# Autodesk Inventor assembly: Intake
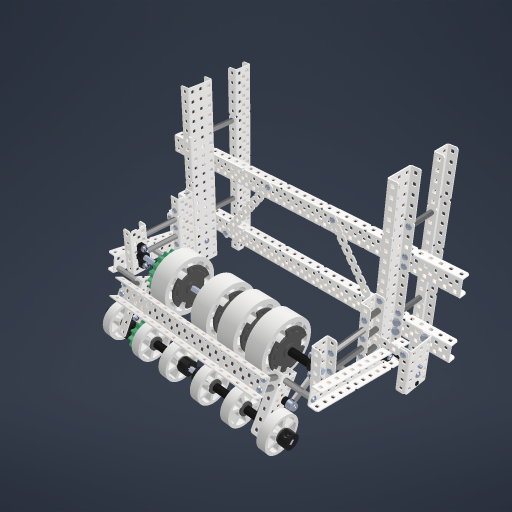
[picture p0: Inventor's stored thumbnail of the model, 512x512]
Saved by Autodesk Inventor 2023 (Build 270158000, 158)
## iProperties
Created: 2022-09-02
Part Number: Intake
Document SubType Name: Assembly
Designer: alex
Author: alex
## Documents named in this file (43)
- C:\Users\alex\Documents\GitHub\4067X_spin_up_cad\Mechanism\Intake.iam
- C:\Users\alex\Documents\GitHub\4067X_spin_up_cad\Library\Structure\Standoff\Standoff 1.00.ipt
- C:\Users\alex\Documents\GitHub\4067X_spin_up_cad\Library\Structure\Standoff.ipt
- C:\Users\alex\Documents\GitHub\4067X_spin_up_cad\Library\Structure\Hardware\Screw Steel - Star\SScrew Star Smooth .290.ipt
- C:\Users\alex\Documents\GitHub\4067X_spin_up_cad\Library\Structure\Hardware\Screw Steel - Star.ipt
- C:\Users\alex\Documents\GitHub\4067X_spin_up_cad\Library\Structure\Standoff\Standoff .50.ipt
- C:\Users\alex\Documents\GitHub\4067X_spin_up_cad\Library\Motion\Spacers\Spacer Nylon .375 OD.ipt
- C:\Users\alex\Documents\GitHub\4067X_spin_up_cad\Library\Structure\Hardware\Nut Keps.ipt
- C:\Users\alex\Documents\GitHub\4067X_spin_up_cad\Library\Structure\Hardware\Screw Steel - Star\SScrew Star Smooth .375.ipt
- C:\Users\alex\Documents\GitHub\4067X_spin_up_cad\Library\Structure\C-Channels\Aluminum 1x3x1\Alu C 1x3x1x20.ipt
- C:\Users\alex\Documents\GitHub\4067X_spin_up_cad\Library\Structure\C-Channels\Aluminum 1x3x1\Alu C 1x3x1x5.ipt
- C:\Users\alex\Documents\GitHub\4067X_spin_up_cad\Library\Structure\C-Channels\Aluminum 1x2x1\Alu C 1x2x1x35.ipt
- C:\Users\alex\Documents\GitHub\4067X_spin_up_cad\Library\Structure\Plates\Aluminum\VEX Plates\Alu Plate VEX 1x11.ipt
- C:\Users\alex\Documents\GitHub\4067X_spin_up_cad\Library\Structure\Standoff\Standoff 2.00.ipt
- C:\Users\alex\Documents\GitHub\4067X_spin_up_cad\Library\Structure\C-Channels\Aluminum 1x2x1\Alu C 1x2x1x5.ipt
- C:\Users\alex\Documents\GitHub\4067X_spin_up_cad\Library\Structure\C-Channels\Aluminum 1x2x1\Alu C 1x2x1x7.ipt
- C:\Users\alex\Documents\GitHub\4067X_spin_up_cad\Library\Structure\Standoff\Standoff .75.ipt
- C:\Users\alex\Documents\GitHub\4067X_spin_up_cad\Library\Motion\Spacers\Spacer Nylon .375 OD\NSpacer .375 OD x .125.ipt
- C:\Users\alex\Documents\GitHub\4067X_spin_up_cad\Library\Motion\Shaft HS\HS Bearing Flat.ipt
- C:\Users\alex\Documents\GitHub\4067X_spin_up_cad\Library\Structure\Hardware\Nut Thin Nylock.ipt
- C:\Users\alex\Documents\GitHub\4067X_spin_up_cad\Library\Structure\Hardware\Screw Steel - Star\SScrew Star Smooth .500.ipt
- C:\Users\alex\Documents\GitHub\4067X_spin_up_cad\Library\Motion\Shaft HS\Shaft HS\Shaft HS 12.0 in.ipt
- C:\Users\alex\Documents\GitHub\4067X_spin_up_cad\Library\Motion\Shaft HS\Shaft HS.ipt
- C:\Users\alex\Documents\GitHub\4067X_spin_up_cad\Library\Motion\Shaft HS\HS Spacer.ipt
- C:\Users\alex\Documents\GitHub\4067X_spin_up_cad\3FlexWheel.iam
- C:\Users\alex\Documents\GitHub\4067X_spin_up_cad\Library\Motion\Shaft HS\HS Spacer\HSpacer .2500.ipt
- C:\Users\alex\Documents\GitHub\4067X_spin_up_cad\Library\Motion\Sprockets\HS 18T Sprocket, No Insert.ipt
- C:\Users\alex\Documents\GitHub\4067X_spin_up_cad\Library\Structure\Hardware\Screw Steel - Star\SScrew Star Smooth 2.250.ipt
- C:\Users\alex\Documents\GitHub\4067X_spin_up_cad\Mechanism\FloatingIntake.iam
- C:\Users\alex\Documents\GitHub\4067X_spin_up_cad\Library\Motion\Spacers\Spacer Nylon .375 OD\NSpacer .375 OD x .375.ipt
- C:\Users\alex\Documents\GitHub\4067X_spin_up_cad\Library\Motion\Spacers\Washer Steel\SWasher .375 OD x .015625.ipt
- C:\Users\alex\Documents\GitHub\4067X_spin_up_cad\Library\Motion\Spacers\Washer Steel.ipt
- C:\Users\alex\Documents\GitHub\4067X_spin_up_cad\Library\Motion\1-Post Bearing Flat Hex Retainer.ipt
- C:\Users\alex\Documents\GitHub\4067X_spin_up_cad\Library\Structure\Hardware\Nut Nylock.ipt
- C:\Users\alex\Documents\GitHub\4067X_spin_up_cad\Library\Motion\Spacers\Spacer Nylon .375 OD\NSpacer .375 OD x .500.ipt
- C:\Users\alex\Documents\GitHub\4067X_spin_up_cad\Library\Motion\Spacers\Washer Teflon\TWasher .375 OD x .06250.ipt
- C:\Users\alex\Documents\GitHub\4067X_spin_up_cad\Library\Motion\Spacers\Washer Teflon.ipt
- C:\Users\alex\Documents\GitHub\4067X_spin_up_cad\Library\Structure\Plates\Aluminum\VEX Plates\Alu Plate VEX 1x4.ipt
- C:\Users\alex\Documents\GitHub\4067X_spin_up_cad\Library\Motion\Shaft HS\HS Shaft Collar.ipt
- C:\Users\alex\Documents\GitHub\4067X_spin_up_cad\Library\Motion\Shaft HS\HS Spacer\HSpacer .5000.ipt
- C:\Users\alex\Documents\GitHub\4067X_spin_up_cad\Library\Motion\Shaft HS\HS Spacer\HSpacer .1250.ipt
- C:\Users\alex\Documents\GitHub\4067X_spin_up_cad\Library\Structure\C-Channels\Aluminum 1x2x1\Alu C 1x2x1x21.ipt
- C:\Users\alex\Documents\GitHub\4067X_spin_up_cad\Library\Structure\Hardware\Screw Steel - Star\SScrew Star Smooth .750.ipt
## Components (157 placed, 35 different names)
1. Alu C 1x3x1x5:1 — Insert:107, Insert:108, Insert:230, Insert:244, Insert:245, Insert:437, Mate:68, Insert:438, Insert:444
2. Alu C 1x2x1x35:1 — Insert:107, Insert:108, Insert:150, Insert:151, Insert:218, Insert:219, Insert:236, Insert:237, Insert:400, Insert:401, Insert:419, Insert:420, Insert:448, Insert:449, Insert:458, Insert:459, Insert:465, Insert:469, Insert:475, Insert:478
3. Standoff 1.00:16 — Insert:110, Insert:404
4. Standoff .50:17 — Insert:110, Insert:496
5. Standoff 1.00:18 — Insert:405
6. Standoff .50:19 — Insert:497
7. Standoff 1.00:20 — Insert:454
8. Standoff .50:21 — Insert:500
9. Standoff 1.00:22 — Insert:455
10. Standoff .50:23 — Insert:501
11. Alu C 1x3x1x5:2 — Insert:150, Insert:151, Insert:217, Insert:220, Insert:221, Insert:428, Mate:67, Insert:429, Insert:439
12. Nut Keps:12 — Insert:217
13. SScrew Star Smooth .290:52 — Insert:218
14. SScrew Star Smooth .290:53 — Insert:219
15. Nut Keps:13 — Insert:220
16. Nut Keps:14 — Insert:221
17. Nut Keps:17 — Insert:230
18. SScrew Star Smooth .290:62 — Insert:236
19. SScrew Star Smooth .290:63 — Insert:237
20. Nut Keps:21 — Insert:244
21. Nut Keps:22 — Insert:245
22. Alu C 1x2x1x35:2 — Insert:417, Insert:418, Insert:466, Insert:467, Insert:470, Insert:476, Insert:477, Insert:481, Insert:482
23. SScrew Star Smooth .290:86 — Insert:456
24. SScrew Star Smooth .290:90 — Insert:407
25. SScrew Star Smooth .290:91 — Insert:406
26. Alu C 1x2x1x5:2 — Insert:334, Insert:335, Insert:338, Insert:339, Insert:488, Mate:72, Insert:489, Insert:490
27. Standoff 2.00:27 — Insert:334, Insert:382
28. Standoff 2.00:28 — Insert:335, Insert:381
29. SScrew Star Smooth .290:102 — Insert:338
30. SScrew Star Smooth .290:103 — Insert:339
31. Alu C 1x2x1x7:1 — Insert:345, Insert:346, Insert:347, Insert:348, Insert:349, Insert:358, Insert:359, Insert:360, Insert:361, Insert:362, Insert:381, Insert:382, Insert:422, Insert:423, Mate:69
32. SScrew Star Smooth .290:106 — Insert:345
33. SScrew Star Smooth .290:107 — Insert:346
34. Standoff .75:29 — Insert:347, Insert:355
35. Standoff .75:30 — Insert:348, Insert:356
36. Standoff .75:31 — Insert:349, Insert:357
37. NSpacer .375 OD x .125:13 — Insert:355
38. NSpacer .375 OD x .125:14 — Insert:356
39. NSpacer .375 OD x .125:15 — Insert:357
40. SScrew Star Smooth .375:111 — Insert:358
41. SScrew Star Smooth .375:112 — Insert:359
42. SScrew Star Smooth .375:113 — Insert:360
43. SScrew Star Smooth .290:114 — Insert:361
44. SScrew Star Smooth .290:115 — Insert:362
45. Alu C 1x2x1x5:3 — Insert:485, Mate:71, Insert:486, Insert:487, Flush:1
46. Standoff 2.00:32 — Insert:384
47. Standoff 2.00:33 — Insert:383
48. SScrew Star Smooth .290:116
49. SScrew Star Smooth .290:117
50. Alu C 1x2x1x7:2 — Insert:383, Insert:384, Insert:402, Insert:403, Mate:70
51. SScrew Star Smooth .290:118
52. SScrew Star Smooth .290:119
53. Standoff .75:34
54. Standoff .75:35
55. Standoff .75:36
56. NSpacer .375 OD x .125:16
57. NSpacer .375 OD x .125:17
58. NSpacer .375 OD x .125:18
59. SScrew Star Smooth .375:120
60. SScrew Star Smooth .375:121
61. SScrew Star Smooth .375:122
62. SScrew Star Smooth .290:123
63. SScrew Star Smooth .290:124
64. Shaft HS 12.0 in:1 — Mate:43, Angle:1, Angle:2, Mate:47, Mate:50, Mate:51, Mate:53, Angle:3, Mate:57, Angle:4, Mate:58, Angle:5, Mate:73, Flush:1, Mate:74
65. 3FlexWheel:1 [sub-assembly] — Mate:43, Angle:1, Mate:48, Mate:76
66. 3FlexWheel:2 [sub-assembly] — Angle:2, Mate:49, Mate:50, Mate:52
67. HSpacer .2500:2 — Mate:47, Mate:48, Mate:49
68. HSpacer .2500:3 — Mate:51, Mate:52, Mate:54
69. 3FlexWheel:3 [sub-assembly] — Mate:53, Angle:3, Mate:54
70. 3FlexWheel:4 [sub-assembly] — Mate:58, Angle:5, Mate:59
71. HS 18T Sprocket, No Insert:1 — Mate:57, Angle:4, Mate:59, Flush:2, Mate:75
72. Alu C 1x3x1x20:3 — Insert:400, Insert:401, Insert:402, Insert:403, Insert:404, Insert:405, Insert:406, Insert:407, Insert:408, Insert:409, Insert:410, Insert:411, Insert:412, Insert:413, Insert:414, Insert:416, Insert:460, Insert:461, Insert:467, Insert:468
73. Nut Keps:41 — Insert:408
74. Nut Keps:42 — Insert:409
75. SScrew Star Smooth .290:129 — Insert:410
76. SScrew Star Smooth .290:130 — Insert:411
77. SScrew Star Smooth .290:131 — Insert:412
78. SScrew Star Smooth 2.250:132 — Insert:413
79. Nut Keps:43 — Insert:414, Insert:433
80. SScrew Star Smooth .290:134 — Insert:416
81. Nut Keps:44 — Insert:417
82. Nut Keps:45 — Insert:418
83. Alu C 1x3x1x20:4 — Insert:419, Insert:420, Insert:421, Insert:422, Insert:423, Insert:424, Mate:66, Insert:446, Insert:450, Insert:451, Insert:452, Insert:453, Insert:454, Insert:455, Insert:456, Insert:457, Insert:462, Insert:463, Insert:464, Insert:479, Insert:480
84. SScrew Star Smooth 2.250:135 — Insert:421, Mate:65
85. Nut Keps:46 — Insert:424, Insert:425
86. FloatingIntake:1 [sub-assembly] — Mate:65, Mate:66, Insert:430, Insert:435, Flush:2
87. NSpacer .375 OD x .375:19 — Insert:425, Insert:426
88. SWasher .375 OD x .015625:1 — Insert:426
89. 1-Post Bearing Flat Hex Retainer:1 — Insert:428, Mate:67
90. Nut Nylock:1
91. SScrew Star Smooth .375:136 — Insert:429
92. NSpacer .375 OD x .500:20 — Insert:430, Insert:431
93. NSpacer .375 OD x .375:21 — Insert:431
94. NSpacer .375 OD x .375:22 — Insert:433
95. SWasher .375 OD x .015625:2
96. NSpacer .375 OD x .500:23 — Insert:435
97. NSpacer .375 OD x .375:24
98. 1-Post Bearing Flat Hex Retainer:2 — Insert:437, Mate:68
99. Nut Nylock:2
100. SScrew Star Smooth .375:137 — Insert:438
101. TWasher .375 OD x .06250:1 — Insert:439, Insert:440
102. Alu Plate VEX 1x4:1 — Insert:440, Mate:69, Insert:441, Insert:447
103. SScrew Star Smooth .375:138 — Insert:441
104. TWasher .375 OD x .06250:2 — Insert:444
105. Alu Plate VEX 1x4:2 — Mate:70
106. SScrew Star Smooth .375:139
107. Nut Keps:47 — Insert:446
108. SScrew Star Smooth .375:140 — Insert:447
109. SScrew Star Smooth .290:141 — Insert:448
110. SScrew Star Smooth .290:142 — Insert:449
111. Nut Keps:48 — Insert:450
112. Nut Keps:49 — Insert:451
113. Nut Keps:50 — Insert:452
114. Nut Keps:51 — Insert:453
115. SScrew Star Smooth .290:143 — Insert:457
116. SScrew Star Smooth .290:144 — Insert:458
117. SScrew Star Smooth .290:145 — Insert:459
118. Nut Keps:52 — Insert:460
119. Nut Keps:53 — Insert:461
120. SScrew Star Smooth .290:146 — Insert:462
121. SScrew Star Smooth .290:147 — Insert:463
122. SScrew Star Smooth .290:148 — Insert:464
123. Alu Plate VEX 1x11:3 — Insert:465, Insert:466, Insert:471, Insert:472
124. SScrew Star Smooth .290:149 — Insert:468
125. Alu Plate VEX 1x11:4 — Insert:469, Insert:470, Insert:473, Insert:474
126. SScrew Star Smooth .290:150 — Insert:471
127. SScrew Star Smooth .290:151 — Insert:472
128. SScrew Star Smooth .290:152 — Insert:473
129. SScrew Star Smooth .290:153 — Insert:474
130. Nut Keps:54 — Insert:475
131. Nut Keps:55 — Insert:476
132. Nut Keps:56 — Insert:477
133. Nut Keps:57 — Insert:478
134. SScrew Star Smooth .290:154 — Insert:479
135. SScrew Star Smooth .290:155 — Insert:480
136. Nut Keps:58 — Insert:481
137. Nut Keps:59 — Insert:482
138. HS Bearing Flat:3 — Insert:485, Mate:71, Insert:493
139. Nut Thin Nylock:5
140. Nut Thin Nylock:6
141. SScrew Star Smooth .500:156 — Insert:486
142. SScrew Star Smooth .500:157 — Insert:487
143. HS Bearing Flat:4 — Insert:488, Mate:72, Mate:73, Insert:491, Insert:492
144. SScrew Star Smooth .500:158 — Insert:489
145. SScrew Star Smooth .500:159 — Insert:490
146. Nut Thin Nylock:7 — Insert:491
147. Nut Thin Nylock:8 — Insert:492
148. HS Shaft Collar:1 — Mate:74, Mate:75
149. HSpacer .5000:4 — Insert:493, Insert:494
150. HSpacer .5000:5 — Insert:494, Insert:495
151. HSpacer .1250:6 — Insert:495, Mate:76
152. Alu C 1x2x1x21:1 — Insert:496, Insert:497, Insert:498, Insert:499
153. SScrew Star Smooth .750:160 — Insert:498
154. SScrew Star Smooth .750:161 — Insert:499
155. Alu C 1x2x1x21:2 — Insert:500, Insert:501, Insert:502, Insert:503
156. SScrew Star Smooth .750:162 — Insert:502
157. SScrew Star Smooth .750:163 — Insert:503
## Relationships (189: Insert 158, Mate 24, Angle 5, Flush 2)
- Insert:107: Alu C 1x3x1x5:1 ↔ Alu C 1x2x1x35:1
- Insert:108: Alu C 1x3x1x5:1 ↔ Alu C 1x2x1x35:1
- Insert:110: Standoff 1.00:16 ↔ Standoff .50:17
- [Insert]: Standoff 1.00:18 ↔ Standoff .50:19
- [Insert]: Standoff 1.00:20 ↔ Standoff .50:21
- [Insert]: Standoff 1.00:22 ↔ Standoff .50:23
- Insert:150: Alu C 1x2x1x35:1 ↔ Alu C 1x3x1x5:2
- Insert:151: Alu C 1x2x1x35:1 ↔ Alu C 1x3x1x5:2
- Insert:217: Alu C 1x3x1x5:2 ↔ Nut Keps:12
- Insert:218: Alu C 1x2x1x35:1 ↔ SScrew Star Smooth .290:52
- Insert:219: Alu C 1x2x1x35:1 ↔ SScrew Star Smooth .290:53
- Insert:220: Alu C 1x3x1x5:2 ↔ Nut Keps:13
- Insert:221: Alu C 1x3x1x5:2 ↔ Nut Keps:14
- Insert:230: Alu C 1x3x1x5:1 ↔ Nut Keps:17
- Insert:236: Alu C 1x2x1x35:1 ↔ SScrew Star Smooth .290:62
- Insert:237: Alu C 1x2x1x35:1 ↔ SScrew Star Smooth .290:63
- Insert:244: Alu C 1x3x1x5:1 ↔ Nut Keps:21
- Insert:245: Alu C 1x3x1x5:1 ↔ Nut Keps:22
- Insert:334: Alu C 1x2x1x5:2 ↔ Standoff 2.00:27
- Insert:335: Alu C 1x2x1x5:2 ↔ Standoff 2.00:28
- Insert:338: Alu C 1x2x1x5:2 ↔ SScrew Star Smooth .290:102
- Insert:339: Alu C 1x2x1x5:2 ↔ SScrew Star Smooth .290:103
- Insert:345: Alu C 1x2x1x7:1 ↔ SScrew Star Smooth .290:106
- Insert:346: Alu C 1x2x1x7:1 ↔ SScrew Star Smooth .290:107
- Insert:347: Alu C 1x2x1x7:1 ↔ Standoff .75:29
- Insert:348: Alu C 1x2x1x7:1 ↔ Standoff .75:30
- Insert:349: Alu C 1x2x1x7:1 ↔ Standoff .75:31
- Insert:355: Standoff .75:29 ↔ NSpacer .375 OD x .125:13
- Insert:356: Standoff .75:30 ↔ NSpacer .375 OD x .125:14
- Insert:357: Standoff .75:31 ↔ NSpacer .375 OD x .125:15
- Insert:358: Alu C 1x2x1x7:1 ↔ SScrew Star Smooth .375:111
- Insert:359: Alu C 1x2x1x7:1 ↔ SScrew Star Smooth .375:112
- Insert:360: Alu C 1x2x1x7:1 ↔ SScrew Star Smooth .375:113
- Insert:361: Alu C 1x2x1x7:1 ↔ SScrew Star Smooth .290:114
- Insert:362: Alu C 1x2x1x7:1 ↔ SScrew Star Smooth .290:115
- [Insert]: Alu C 1x2x1x5:3 ↔ Standoff 2.00:32
- [Insert]: Alu C 1x2x1x5:3 ↔ Standoff 2.00:33
- [Insert]: Alu C 1x2x1x5:3 ↔ SScrew Star Smooth .290:116
- [Insert]: Alu C 1x2x1x5:3 ↔ SScrew Star Smooth .290:117
- [Insert]: Alu C 1x2x1x7:2 ↔ SScrew Star Smooth .290:118
- [Insert]: Alu C 1x2x1x7:2 ↔ SScrew Star Smooth .290:119
- [Insert]: Alu C 1x2x1x7:2 ↔ Standoff .75:34
- [Insert]: Alu C 1x2x1x7:2 ↔ Standoff .75:35
- [Insert]: Alu C 1x2x1x7:2 ↔ Standoff .75:36
- [Insert]: Standoff .75:34 ↔ NSpacer .375 OD x .125:16
- [Insert]: Standoff .75:35 ↔ NSpacer .375 OD x .125:17
- [Insert]: Standoff .75:36 ↔ NSpacer .375 OD x .125:18
- [Insert]: Alu C 1x2x1x7:2 ↔ SScrew Star Smooth .375:120
- [Insert]: Alu C 1x2x1x7:2 ↔ SScrew Star Smooth .375:121
- [Insert]: Alu C 1x2x1x7:2 ↔ SScrew Star Smooth .375:122
- [Insert]: Alu C 1x2x1x7:2 ↔ SScrew Star Smooth .290:123
- [Insert]: Alu C 1x2x1x7:2 ↔ SScrew Star Smooth .290:124
- Insert:381: Standoff 2.00:28 ↔ Alu C 1x2x1x7:1
- Insert:382: Standoff 2.00:27 ↔ Alu C 1x2x1x7:1
- Insert:383: Standoff 2.00:33 ↔ Alu C 1x2x1x7:2
- Insert:384: Standoff 2.00:32 ↔ Alu C 1x2x1x7:2
- Mate:43: Shaft HS 12.0 in:1 ↔ 3FlexWheel:1
- Angle:1 (0 deg): Shaft HS 12.0 in:1 ↔ 3FlexWheel:1
- Angle:2 (0 deg): Shaft HS 12.0 in:1 ↔ 3FlexWheel:2
- Mate:47: Shaft HS 12.0 in:1 ↔ HSpacer .2500:2
- Mate:48: 3FlexWheel:1 ↔ HSpacer .2500:2
- Mate:49: 3FlexWheel:2 ↔ HSpacer .2500:2
- Mate:50: Shaft HS 12.0 in:1 ↔ 3FlexWheel:2
- Mate:51: Shaft HS 12.0 in:1 ↔ HSpacer .2500:3
- Mate:52: 3FlexWheel:2 ↔ HSpacer .2500:3
- Mate:53: Shaft HS 12.0 in:1 ↔ 3FlexWheel:3
- Angle:3 (0 deg): Shaft HS 12.0 in:1 ↔ 3FlexWheel:3
- Mate:54: HSpacer .2500:3 ↔ 3FlexWheel:3
- Mate:57: Shaft HS 12.0 in:1 ↔ HS 18T Sprocket, No Insert:1
- Angle:4 (0 deg): Shaft HS 12.0 in:1 ↔ HS 18T Sprocket, No Insert:1
- Mate:58: Shaft HS 12.0 in:1 ↔ 3FlexWheel:4
- Angle:5 (0 deg): Shaft HS 12.0 in:1 ↔ 3FlexWheel:4
- Mate:59: 3FlexWheel:4 ↔ HS 18T Sprocket, No Insert:1
- Insert:400: Alu C 1x2x1x35:1 ↔ Alu C 1x3x1x20:3
- Insert:401: Alu C 1x2x1x35:1 ↔ Alu C 1x3x1x20:3
- Insert:402: Alu C 1x2x1x7:2 ↔ Alu C 1x3x1x20:3
- Insert:403: Alu C 1x2x1x7:2 ↔ Alu C 1x3x1x20:3
- Insert:404: Standoff 1.00:16 ↔ Alu C 1x3x1x20:3
- Insert:405: Standoff 1.00:18 ↔ Alu C 1x3x1x20:3
- Insert:406: SScrew Star Smooth .290:91 ↔ Alu C 1x3x1x20:3
- Insert:407: SScrew Star Smooth .290:90 ↔ Alu C 1x3x1x20:3
- Insert:408: Alu C 1x3x1x20:3 ↔ Nut Keps:41
- Insert:409: Alu C 1x3x1x20:3 ↔ Nut Keps:42
- Insert:410: Alu C 1x3x1x20:3 ↔ SScrew Star Smooth .290:129
- Insert:411: Alu C 1x3x1x20:3 ↔ SScrew Star Smooth .290:130
- Insert:412: Alu C 1x3x1x20:3 ↔ SScrew Star Smooth .290:131
- Insert:413: Alu C 1x3x1x20:3 ↔ SScrew Star Smooth 2.250:132
- Insert:414: Alu C 1x3x1x20:3 ↔ Nut Keps:43
- Insert:416: Alu C 1x3x1x20:3 ↔ SScrew Star Smooth .290:134
- Insert:417: Alu C 1x2x1x35:2 ↔ Nut Keps:44
- Insert:418: Alu C 1x2x1x35:2 ↔ Nut Keps:45
- Insert:419: Alu C 1x2x1x35:1 ↔ Alu C 1x3x1x20:4
- Insert:420: Alu C 1x2x1x35:1 ↔ Alu C 1x3x1x20:4
- Insert:421: Alu C 1x3x1x20:4 ↔ SScrew Star Smooth 2.250:135
- Insert:422: Alu C 1x2x1x7:1 ↔ Alu C 1x3x1x20:4
- Insert:423: Alu C 1x2x1x7:1 ↔ Alu C 1x3x1x20:4
- Insert:424: Alu C 1x3x1x20:4 ↔ Nut Keps:46
- Mate:65: SScrew Star Smooth 2.250:135 ↔ FloatingIntake:1
- Mate:66 (13.6398 mm): Alu C 1x3x1x20:4 ↔ FloatingIntake:1
- Insert:425: Nut Keps:46 ↔ NSpacer .375 OD x .375:19
- Insert:426: NSpacer .375 OD x .375:19 ↔ SWasher .375 OD x .015625:1
- [Insert]: 1-Post Bearing Flat Hex Retainer:1 ↔ Nut Nylock:1
- Insert:428: Alu C 1x3x1x5:2 ↔ 1-Post Bearing Flat Hex Retainer:1
- Mate:67: Alu C 1x3x1x5:2 ↔ 1-Post Bearing Flat Hex Retainer:1
- Insert:429: Alu C 1x3x1x5:2 ↔ SScrew Star Smooth .375:136
- Insert:430: FloatingIntake:1 ↔ NSpacer .375 OD x .500:20
- Insert:431: NSpacer .375 OD x .500:20 ↔ NSpacer .375 OD x .375:21
- [Insert]: NSpacer .375 OD x .375:22 ↔ SWasher .375 OD x .015625:2
- Insert:433: Nut Keps:43 ↔ NSpacer .375 OD x .375:22
- [Insert]: NSpacer .375 OD x .500:23 ↔ NSpacer .375 OD x .375:24
- Insert:435: FloatingIntake:1 ↔ NSpacer .375 OD x .500:23
- [Insert]: 1-Post Bearing Flat Hex Retainer:2 ↔ Nut Nylock:2
- Insert:437: Alu C 1x3x1x5:1 ↔ 1-Post Bearing Flat Hex Retainer:2
- Mate:68: Alu C 1x3x1x5:1 ↔ 1-Post Bearing Flat Hex Retainer:2
- Insert:438: Alu C 1x3x1x5:1 ↔ SScrew Star Smooth .375:137
- Insert:439: Alu C 1x3x1x5:2 ↔ TWasher .375 OD x .06250:1
- Insert:440: TWasher .375 OD x .06250:1 ↔ Alu Plate VEX 1x4:1
- Mate:69: Alu C 1x2x1x7:1 ↔ Alu Plate VEX 1x4:1
- Insert:441: Alu Plate VEX 1x4:1 ↔ SScrew Star Smooth .375:138
- [Insert]: TWasher .375 OD x .06250:2 ↔ Alu Plate VEX 1x4:2
- [Insert]: Alu Plate VEX 1x4:2 ↔ SScrew Star Smooth .375:139
- Insert:444: Alu C 1x3x1x5:1 ↔ TWasher .375 OD x .06250:2
- Mate:70: Alu C 1x2x1x7:2 ↔ Alu Plate VEX 1x4:2
- Insert:446: Alu C 1x3x1x20:4 ↔ Nut Keps:47
- Insert:447: Alu Plate VEX 1x4:1 ↔ SScrew Star Smooth .375:140
- Insert:448: Alu C 1x2x1x35:1 ↔ SScrew Star Smooth .290:141
- Insert:449: Alu C 1x2x1x35:1 ↔ SScrew Star Smooth .290:142
- Insert:450: Alu C 1x3x1x20:4 ↔ Nut Keps:48
- Insert:451: Alu C 1x3x1x20:4 ↔ Nut Keps:49
- Insert:452: Alu C 1x3x1x20:4 ↔ Nut Keps:50
- Insert:453: Alu C 1x3x1x20:4 ↔ Nut Keps:51
- Insert:454: Standoff 1.00:20 ↔ Alu C 1x3x1x20:4
- Insert:455: Standoff 1.00:22 ↔ Alu C 1x3x1x20:4
- Insert:456: SScrew Star Smooth .290:86 ↔ Alu C 1x3x1x20:4
- Insert:457: Alu C 1x3x1x20:4 ↔ SScrew Star Smooth .290:143
- Insert:458: Alu C 1x2x1x35:1 ↔ SScrew Star Smooth .290:144
- Insert:459: Alu C 1x2x1x35:1 ↔ SScrew Star Smooth .290:145
- Insert:460: Alu C 1x3x1x20:3 ↔ Nut Keps:52
- Insert:461: Alu C 1x3x1x20:3 ↔ Nut Keps:53
- Insert:462: Alu C 1x3x1x20:4 ↔ SScrew Star Smooth .290:146
- Insert:463: Alu C 1x3x1x20:4 ↔ SScrew Star Smooth .290:147
- Insert:464: Alu C 1x3x1x20:4 ↔ SScrew Star Smooth .290:148
- Insert:465: Alu C 1x2x1x35:1 ↔ Alu Plate VEX 1x11:3
- Insert:466: Alu C 1x2x1x35:2 ↔ Alu Plate VEX 1x11:3
- Insert:467: Alu C 1x2x1x35:2 ↔ Alu C 1x3x1x20:3
- Insert:468: Alu C 1x3x1x20:3 ↔ SScrew Star Smooth .290:149
- Insert:469: Alu C 1x2x1x35:1 ↔ Alu Plate VEX 1x11:4
- Insert:470: Alu C 1x2x1x35:2 ↔ Alu Plate VEX 1x11:4
- Insert:471: Alu Plate VEX 1x11:3 ↔ SScrew Star Smooth .290:150
- Insert:472: Alu Plate VEX 1x11:3 ↔ SScrew Star Smooth .290:151
- Insert:473: Alu Plate VEX 1x11:4 ↔ SScrew Star Smooth .290:152
- Insert:474: Alu Plate VEX 1x11:4 ↔ SScrew Star Smooth .290:153
- Insert:475: Alu C 1x2x1x35:1 ↔ Nut Keps:54
- Insert:476: Alu C 1x2x1x35:2 ↔ Nut Keps:55
- Insert:477: Alu C 1x2x1x35:2 ↔ Nut Keps:56
- Insert:478: Alu C 1x2x1x35:1 ↔ Nut Keps:57
- Insert:479: Alu C 1x3x1x20:4 ↔ SScrew Star Smooth .290:154
- Insert:480: Alu C 1x3x1x20:4 ↔ SScrew Star Smooth .290:155
- Insert:481: Alu C 1x2x1x35:2 ↔ Nut Keps:58
- Insert:482: Alu C 1x2x1x35:2 ↔ Nut Keps:59
- [Insert]: HS Bearing Flat:3 ↔ Nut Thin Nylock:5
- [Insert]: HS Bearing Flat:3 ↔ Nut Thin Nylock:6
- Insert:485: Alu C 1x2x1x5:3 ↔ HS Bearing Flat:3
- Mate:71: Alu C 1x2x1x5:3 ↔ HS Bearing Flat:3
- Insert:486: Alu C 1x2x1x5:3 ↔ SScrew Star Smooth .500:156
- Insert:487: Alu C 1x2x1x5:3 ↔ SScrew Star Smooth .500:157
- Insert:488: Alu C 1x2x1x5:2 ↔ HS Bearing Flat:4
- Mate:72: Alu C 1x2x1x5:2 ↔ HS Bearing Flat:4
- Insert:489: Alu C 1x2x1x5:2 ↔ SScrew Star Smooth .500:158
- Insert:490: Alu C 1x2x1x5:2 ↔ SScrew Star Smooth .500:159
- Mate:73: Shaft HS 12.0 in:1 ↔ HS Bearing Flat:4
- Insert:491: HS Bearing Flat:4 ↔ Nut Thin Nylock:7
- Insert:492: HS Bearing Flat:4 ↔ Nut Thin Nylock:8
- Flush:1 (-6.0198 mm): Alu C 1x2x1x5:3 ↔ Shaft HS 12.0 in:1
- Flush:2: HS 18T Sprocket, No Insert:1 ↔ FloatingIntake:1
- Mate:74: Shaft HS 12.0 in:1 ↔ HS Shaft Collar:1
- Mate:75: HS 18T Sprocket, No Insert:1 ↔ HS Shaft Collar:1
- Insert:493: HS Bearing Flat:3 ↔ HSpacer .5000:4
- Insert:494: HSpacer .5000:4 ↔ HSpacer .5000:5
- Insert:495: HSpacer .5000:5 ↔ HSpacer .1250:6
- Mate:76: 3FlexWheel:1 ↔ HSpacer .1250:6
- Insert:496: Standoff .50:17 ↔ Alu C 1x2x1x21:1
- Insert:497: Standoff .50:19 ↔ Alu C 1x2x1x21:1
- Insert:498: Alu C 1x2x1x21:1 ↔ SScrew Star Smooth .750:160
- Insert:499: Alu C 1x2x1x21:1 ↔ SScrew Star Smooth .750:161
- Insert:500: Standoff .50:21 ↔ Alu C 1x2x1x21:2
- Insert:501: Standoff .50:23 ↔ Alu C 1x2x1x21:2
- Insert:502: Alu C 1x2x1x21:2 ↔ SScrew Star Smooth .750:162
- Insert:503: Alu C 1x2x1x21:2 ↔ SScrew Star Smooth .750:163
## Named parameters: d171_d169 = 0 mm, d195_d169 = 0 mm, d197_d195_d169 = 0 mm, d492_d477 = 0 mm, d493_d478 = 0 mm, d494_d484 = 0 mm, d495_d485 = 0 mm, d496_d486 = 0 mm, d497_d487 = 0 mm, d498_d488 = 0 mm, d499_d489 = 0 mm, d500_d490 = 0 mm, d501_d491 = 0 mm, d502_d463 = 0 mm, d503_d464 = 0 mm, d504_d467 = 0 mm, d505_d468 = 0 mm, d506_d474 = 0 mm, d507_d475 = 0 mm, d508_d476 = 0 mm, d208_d147 = 0 mm, d606_d599 = 0 mm, d608_d605 = 0 mm, d610_d208_d147 = 0 mm, d618_d615 = 0 mm, d619_d617 = 0 mm, d660_d521_d253_d244 = 0 mm, d661_d522_d520 = 0 mm
